# Autodesk Inventor assembly: cabinet
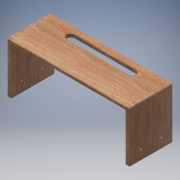
[picture p0: Inventor's stored thumbnail of the model, 180x180]
Saved by Autodesk Inventor 2016 (Build 200138000, 138)
## iProperties
Created: 2015-10-24
Part Number: cabinet
Document SubType Name: Assembly
Designer: jeremyhale
Mass: 6489.05 g
Surface Area: 8255.95 cm^2
Volume: 6489.05 cm^3
Density: 1 g/cm^3
Author: jeremyhale
## Documents named in this file (4)
- \\psf\Home\Documents\Poorhouse\git\p0001\cabinet.iam
- \\psf\Home\Documents\Poorhouse\git\p0001\cabinet-side.ipt
- \\psf\Home\Documents\Poorhouse\git\p0001\cabinet-top.ipt
- \\psf\Home\Documents\Poorhouse\git\p0001\cabinet-side_MIR.ipt
## Components (3 placed, 3 different names)
1. cabinet-side:1 — Rigid:2
2. top — Rigid:2
3. cabinet-side_MIR:1
## Relationships (1: WeldJoint 1)
- Rigid:2 [WeldJoint]: cabinet-side:1 ↔ top
